# Autodesk Inventor assembly: 288635
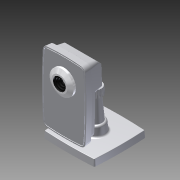
[picture p0: Inventor's stored thumbnail of the model, 180x180]
Saved by Autodesk Inventor 2012 (Build 160160000, 160)
## iProperties
Category: Control System
Company: Autodesk Inc.
Created: 2012-01-03
Part Number: 288635
Document SubType Name: Assembly
Designer: Autodesk Inc.
Catalog Web Link: http://www.axis.com/products/cam_m1011/
Description: Camera
Vendor: Axis
Author: Autodesk Inc.
## Documents named in this file (3)
- C:\Data Folder\FIRST 2012\KOP\All Parts 2012\Control System\ControlSystem_Camera_Axis_288635.iam
- C:\Data Folder\FIRST 2012\KOP\All Parts 2012\Miscellaneous\ControlSystem_Camera_Axis_M1011_Base.ipt
- C:\Data Folder\FIRST 2012\KOP\All Parts 2012\Control System\ControlSystem_Camera_Axis_Camera.ipt
## Components (2 placed, 2 different names)
1. ControlSystem_Camera_Axis_M1011_Base:1 — Flush:2, Mate:1, Tangent:1, Tangent:2
2. ControlSystem_Camera_Axis_Camera:1 — Mate:1, Tangent:1, Tangent:2
## Relationships (4: Tangent 2, Flush 1, Mate 1)
- Flush:2 (-4.7625 mm): ControlSystem_Camera_Axis_M1011_Base:1
- Mate:1: ControlSystem_Camera_Axis_M1011_Base:1 ↔ ControlSystem_Camera_Axis_Camera:1
- Tangent:1: ControlSystem_Camera_Axis_M1011_Base:1 ↔ ControlSystem_Camera_Axis_Camera:1
- Tangent:2: ControlSystem_Camera_Axis_M1011_Base:1 ↔ ControlSystem_Camera_Axis_Camera:1
